# Autodesk Inventor assembly: OutputShaft
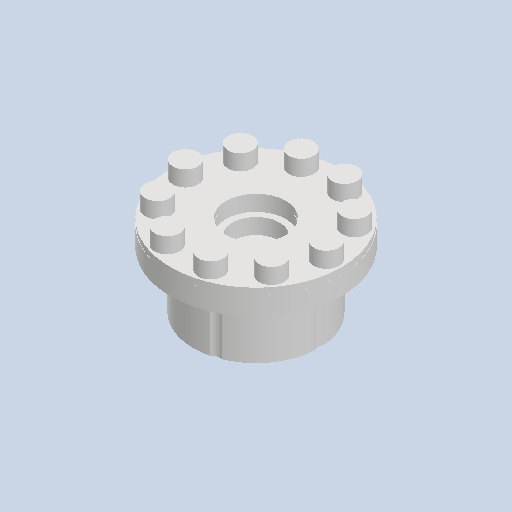
[picture p0: Inventor's stored thumbnail of the model, 512x512]
Saved by Autodesk Inventor 2022 (Build 260153000, 153)
## iProperties
Created: 2022-10-09
Part Number: OutputShaft
Document SubType Name: Assembly
Designer: MicnedSQ
Author: MicnedSQ
## Documents named in this file (3)
- C:\Users\Micne\Desktop\RobotArmV1\RotatingBase\CycloidalDrive\OutputShaft.iam
- C:\Users\Micne\Desktop\RobotArmV1\RotatingBase\CycloidalDrive\OutputShaft1.ipt
- C:\Users\Micne\Desktop\RobotArmV1\RotatingBase\CycloidalDrive\OutputShaft2.ipt
## Components (2 placed, 2 different names)
1. OutputShaft1:1 — Sztywne:1
2. OutputShaft2:1 — Sztywne:1
## Relationships (1: WeldJoint 1)
- Sztywne:1 [WeldJoint]: OutputShaft1:1 ↔ OutputShaft2:1
